# Autodesk Inventor assembly: COXA_UNIT_ASM
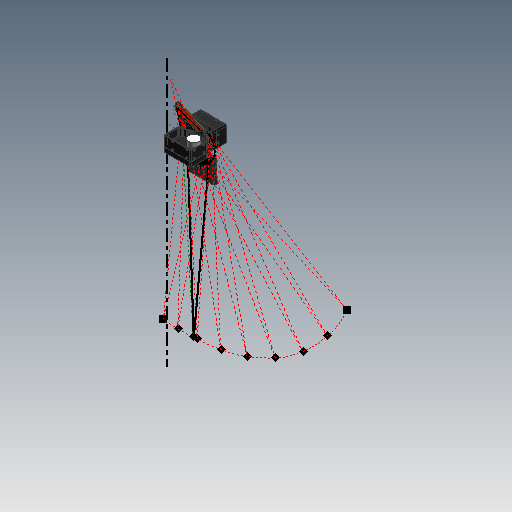
[picture p0: Inventor's stored thumbnail of the model, 512x512]
Saved by Autodesk Inventor 2019.4 (Build 234330000, 330)
## iProperties
Created: 2019-10-21
Part Number: COXA_UNIT_ASM
Material: 一般
Document SubType Name: Assembly
Designer: y6tada
Author: y6tada
## Documents named in this file (7)
- C:\Workspace\Yuni9\Inventor\Asm\COXA_UNIT\COXA_UNIT_ASM.iam
- C:\Workspace\Yuni9\Inventor\Libs\DYNAMIXEL\XM430\XM430_ASM_WITHOUT-BACK.iam
- C:\Workspace\Yuni9\Inventor\Asm\COXA_UNIT\COXA_YAW_SERVO_BASE.ipt
- C:\Workspace\Yuni9\Inventor\Asm\COXA_UNIT\COXA_YAW_SUPPORT-LINK_BACK.ipt
- C:\Workspace\Yuni9\Inventor\Asm\COXA_UNIT\COXA_ROLL_SERVO-OUTPUT.ipt
- C:\Workspace\Yuni9\Inventor\Asm\COXA_UNIT\COXA_ROLL_LONG-LINK.ipt
- C:\Workspace\Yuni9\Inventor\Asm\COXA_UNIT\COXA_ROLL_COUPLER_BACK.ipt
## Components (7 placed, 6 different names)
1. XM430_ASM_WITHOUT-BACK:1 [sub-assembly] — メイト:1, フラッシュ:3, 角度:2, メイト:20, メイト:21, メイト:22
2. XM430_ASM_WITHOUT-BACK:2 [sub-assembly] — メイト:7, 角度:2
3. COXA_YAW_SERVO_BASE:1 — フラッシュ:1, メイト:6, メイト:8, メイト:11, メイト:20, メイト:21, メイト:22
4. COXA_YAW_SUPPORT-LINK_BACK:1 — メイト:8, メイト:11, メイト:13, メイト:14, メイト:15, メイト:16
5. COXA_ROLL_SERVO-OUTPUT:1 — メイト:12, メイト:13, メイト:14, メイト:17, メイト:18
6. COXA_ROLL_LONG-LINK:1 — メイト:15, メイト:16, メイト:19
7. COXA_ROLL_COUPLER_BACK:1 — メイト:17, メイト:18, メイト:19
## Relationships (20: Mate 16, Flush 2, Angle 2)
- メイト:1 [Mate] (25 mm): XM430_ASM_WITHOUT-BACK:1
- フラッシュ:3 [Flush]: XM430_ASM_WITHOUT-BACK:1
- フラッシュ:1 [Flush]: COXA_YAW_SERVO_BASE:1
- メイト:6 [Mate]: COXA_YAW_SERVO_BASE:1
- 角度:1 [Angle] (0 deg)
- メイト:7 [Mate]: XM430_ASM_WITHOUT-BACK:2
- 角度:2 [Angle] (0 deg): XM430_ASM_WITHOUT-BACK:1 ↔ XM430_ASM_WITHOUT-BACK:2
- メイト:8 [Mate]: COXA_YAW_SERVO_BASE:1 ↔ COXA_YAW_SUPPORT-LINK_BACK:1
- メイト:11 [Mate]: COXA_YAW_SERVO_BASE:1 ↔ COXA_YAW_SUPPORT-LINK_BACK:1
- メイト:12 [Mate]: COXA_ROLL_SERVO-OUTPUT:1
- メイト:13 [Mate]: COXA_YAW_SUPPORT-LINK_BACK:1 ↔ COXA_ROLL_SERVO-OUTPUT:1
- メイト:14 [Mate]: COXA_YAW_SUPPORT-LINK_BACK:1 ↔ COXA_ROLL_SERVO-OUTPUT:1
- メイト:15 [Mate]: COXA_YAW_SUPPORT-LINK_BACK:1 ↔ COXA_ROLL_LONG-LINK:1
- メイト:16 [Mate]: COXA_YAW_SUPPORT-LINK_BACK:1 ↔ COXA_ROLL_LONG-LINK:1
- メイト:17 [Mate]: COXA_ROLL_SERVO-OUTPUT:1 ↔ COXA_ROLL_COUPLER_BACK:1
- メイト:18 [Mate]: COXA_ROLL_SERVO-OUTPUT:1 ↔ COXA_ROLL_COUPLER_BACK:1
- メイト:19 [Mate]: COXA_ROLL_LONG-LINK:1 ↔ COXA_ROLL_COUPLER_BACK:1
- メイト:20 [Mate]: XM430_ASM_WITHOUT-BACK:1 ↔ COXA_YAW_SERVO_BASE:1
- メイト:21 [Mate]: XM430_ASM_WITHOUT-BACK:1 ↔ COXA_YAW_SERVO_BASE:1
- メイト:22 [Mate]: XM430_ASM_WITHOUT-BACK:1 ↔ COXA_YAW_SERVO_BASE:1
